# Autodesk Inventor assembly: 3.25 Traction AS, Circle_MIR
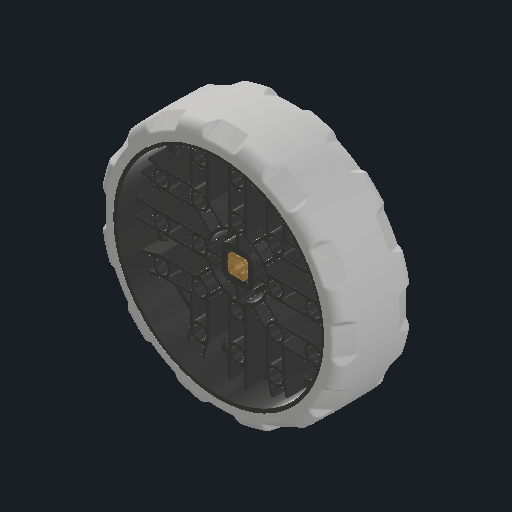
[picture p0: Inventor's stored thumbnail of the model, 512x512]
Saved by Autodesk Inventor 2026.2 (Build 302298000, 298)
## iProperties
Created: 2022-08-02
Part Number: 3.25 Traction AS, Circle_MIR
Document SubType Name: Assembly
Designer: sakin_wbdzdu1
Author: ylu12
## Documents named in this file (3)
- C:\Personal\Deprecated\VEX V5 Push Back\S-bot-two\CAD\VEX-CAD-Inventor-1.4.2\Motion\Wheels\Traction Wheel\3.25 Traction AS, Circle_MIR.iam
- C:\Personal\Deprecated\VEX V5 Push Back\S-bot-two\CAD\VEX-CAD-Inventor-1.4.2\Motion\Wheels\Reference Files\3.25 Traction Antistatic_MIR.ipt
- C:\Personal\Deprecated\VEX V5 Push Back\S-bot-two\CAD\VEX-CAD-Inventor-1.4.2\Motion\HS Shaft Adapter Circle_MIR.ipt
## Components (2 placed, 2 different names)
1. 3.25 Traction Antistatic_MIR:1 — Mate:24, Mate:22, Mate:20
2. HS Shaft Adapter Circle_MIR:1 — Flush:10, Mate:33, Mate:32
## Relationships (6: Flush 3, Mate 3)
- Mate:24 [Flush]: 3.25 Traction Antistatic_MIR:1
- Mate:22 [Flush]: 3.25 Traction Antistatic_MIR:1
- Mate:20: 3.25 Traction Antistatic_MIR:1
- Flush:10 (-6.35 mm): HS Shaft Adapter Circle_MIR:1
- Mate:33: HS Shaft Adapter Circle_MIR:1
- Mate:32: HS Shaft Adapter Circle_MIR:1
## Named parameters: Thickness = 8.255 mm
